# Autodesk Inventor assembly: 3826_2013_Bumpers copy
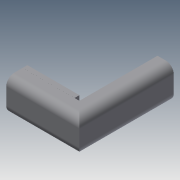
[picture p0: Inventor's stored thumbnail of the model, 180x180]
Saved by Autodesk Inventor 2015 (Build 190159000, 159)
## iProperties
Created: 2013-02-04
Part Number: 3826_2013_Bumpers copy
Document SubType Name: Assembly
Designer: Joshua
Author: Joshua
## Documents named in this file (4)
- C:\Users\Joshua\Documents\3826 For Life!\CAD\3826-2016\Robot\3826_2013_Bumpers copy.iam
- C:\Users\Joshua\Documents\3826 For Life!\CAD\3826_2013\Part50.ipt
- C:\Users\Joshua\Documents\3826 For Life!\CAD\3826_2013\Part52.ipt
- C:\Users\Joshua\Documents\3826 For Life!\CAD\3826_2013\Part53.ipt
## Components (3 placed, 3 different names)
1. Part50:1 — Mate:2, Flush:3, Flush:6
2. Part52:1 — Mate:2, Flush:3, Flush:6
3. Part53:1
## Relationships (3: Flush 2, Mate 1)
- Mate:2: Part50:1 ↔ Part52:1
- Flush:3: Part50:1 ↔ Part52:1
- Flush:6: Part50:1 ↔ Part52:1
